# Autodesk Inventor assembly: LowerLeg
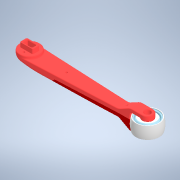
[picture p0: Inventor's stored thumbnail of the model, 180x180]
Saved by Autodesk Inventor 2022.2 (Build 262287000, 287)
## iProperties
Created: 2021-12-29
Part Number: LowerLeg
Document SubType Name: Assembly
Designer: Jochen
Author: Jochen
## Documents named in this file (3)
- D:\Projects\Lisbeth\CAD\LowerLeg\LowerLeg.iam
- D:\Projects\Lisbeth\CAD\LowerLeg\LowerLegBody.ipt
- D:\Projects\Lisbeth\CAD\foot\Foot.iam
## Components (2 placed, 2 different names)
1. LowerLegBody:1 — Mate:1, Mate:2, Mate:3, Mate:4, Mate:5, Mate:6
2. Foot:1 [sub-assembly] — Mate:4, Mate:5, Mate:6
## Relationships (6: Mate 6)
- Mate:1: LowerLegBody:1
- Mate:2: LowerLegBody:1
- Mate:3: LowerLegBody:1
- Mate:4: LowerLegBody:1 ↔ Foot:1
- Mate:5: LowerLegBody:1 ↔ Foot:1
- Mate:6: LowerLegBody:1 ↔ Foot:1
